# Autodesk Inventor assembly: CamLeft
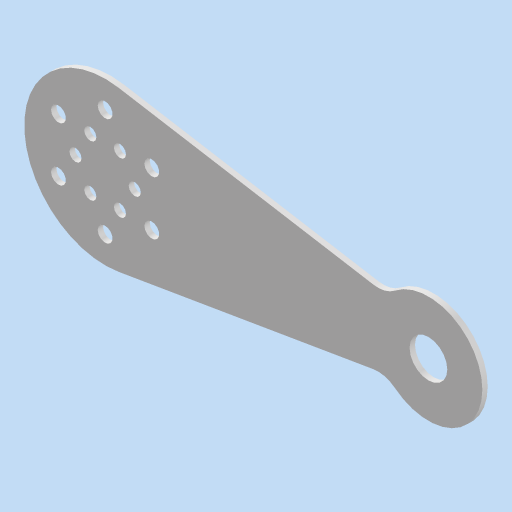
[picture p0: Inventor's stored thumbnail of the model, 512x512]
Saved by Autodesk Inventor 2023 (Build 270158000, 158)
## iProperties
Created: 2026-05-26
Part Number: CamLeft
Document SubType Name: Assembly
Designer: Nathann
Author: Nathann
Revision Number: ANY
## iProperties of the stored document MemberDocs/xCvynumyaGsfmvgzwCpa1trsjKb
Created: 2026-05-26
Part Number: CamLeft
Document SubType Name: Assembly
Designer: Nathann
Author: Nathann
Revision Number: ANY
## Documents named in this file (56)
- C:\Users\Nathann\OneDrive\ClawdDrive\Objet3D\RunningRobot\PartURDF\CamLeft.iam
- C:\Users\Nathann\OneDrive\ClawdDrive\Objet3D\RunningRobot\testfour_bar_bend_Défaut.ipt
- C:\Users\Nathann\OneDrive\ClawdDrive\Objet3D\RunningRobot\testChassis Connector.ipt
- C:\Users\Nathann\OneDrive\ClawdDrive\Objet3D\RunningRobot\testHip Hinge Base.ipt
- C:\Users\Nathann\OneDrive\ClawdDrive\Objet3D\RunningRobot\testHip Hinge Base 2.ipt
- C:\Users\Nathann\OneDrive\ClawdDrive\Objet3D\RunningRobot\testHip Motor Connector.ipt
- C:\Users\Nathann\OneDrive\ClawdDrive\Objet3D\RunningRobot\testAdduction Base.ipt
- C:\Users\Nathann\OneDrive\ClawdDrive\Objet3D\RunningRobot\testAK-60 Phantom_Défaut_1.iam
- C:\Users\Nathann\OneDrive\ClawdDrive\Objet3D\RunningRobot\testAKE90-8-KV35.ipt
- C:\Users\Nathann\OneDrive\ClawdDrive\Objet3D\RunningRobot\testDriver Placeholder.ipt
- C:\Users\Nathann\OneDrive\ClawdDrive\Objet3D\RunningRobot\testfour_bar_hip_adapter_Défaut.ipt
- C:\Users\Nathann\OneDrive\ClawdDrive\Objet3D\RunningRobot\testCFRP Tube Attachment Male Left.ipt
- C:\Users\Nathann\OneDrive\ClawdDrive\Objet3D\RunningRobot\testCFRP Tube Attachment Female_Défaut.ipt
- C:\Users\Nathann\OneDrive\ClawdDrive\Objet3D\RunningRobot\testigus adapter_Défaut.ipt
- C:\Users\Nathann\OneDrive\ClawdDrive\Objet3D\RunningRobot\testJFM-0810-05.ipt
- C:\Users\Nathann\OneDrive\ClawdDrive\Objet3D\RunningRobot\testJTM-0818-015.ipt
- C:\Users\Nathann\OneDrive\ClawdDrive\Objet3D\RunningRobot\testCFRP Tube_Défaut.ipt
- C:\Users\Nathann\OneDrive\ClawdDrive\Objet3D\RunningRobot\testCFRP Tube Attachment Male_Défaut.ipt
- C:\Users\Nathann\OneDrive\ClawdDrive\Objet3D\RunningRobot\testfour_bar_knee_adapter_Défaut.ipt
- C:\Users\Nathann\OneDrive\ClawdDrive\Objet3D\RunningRobot\testCFRP Tube Plug_Défaut.ipt
- C:\Users\Nathann\OneDrive\ClawdDrive\Objet3D\RunningRobot\testUpper Leg Plate_Défaut.ipt
- C:\Users\Nathann\OneDrive\ClawdDrive\Objet3D\RunningRobot\testUpper Leg Spacer_Défaut.ipt
- C:\Users\Nathann\OneDrive\ClawdDrive\Objet3D\RunningRobot\testMotor Adapter Plate_Défaut.ipt
- C:\Users\Nathann\OneDrive\ClawdDrive\Objet3D\RunningRobot\testKnee Joint Outer_Défaut.ipt
- C:\Users\Nathann\OneDrive\ClawdDrive\Objet3D\RunningRobot\testknee bearing holder_Défaut.ipt
- C:\Users\Nathann\OneDrive\ClawdDrive\Objet3D\RunningRobot\testShin_Spacer_Défaut.ipt
- C:\Users\Nathann\OneDrive\ClawdDrive\Objet3D\RunningRobot\testShin_Plate_Défaut.ipt
- C:\Users\Nathann\OneDrive\ClawdDrive\Objet3D\RunningRobot\testAchilles Base_Défaut.ipt
- C:\Users\Nathann\OneDrive\ClawdDrive\Objet3D\RunningRobot\testAchilles Joint_Défaut.ipt
- C:\Users\Nathann\OneDrive\ClawdDrive\Objet3D\RunningRobot\testWasher M8 ISO 7089 ALU_Défaut.ipt
- C:\Users\Nathann\OneDrive\ClawdDrive\Objet3D\RunningRobot\testNETW6.ipt
- C:\Users\Nathann\OneDrive\ClawdDrive\Objet3D\RunningRobot\testNut M8 ISO 4032_Défaut.ipt
- C:\Users\Nathann\OneDrive\ClawdDrive\Objet3D\RunningRobot\testEST-221-Durovis_EST-221-Durovis.ipt
- C:\Users\Nathann\OneDrive\ClawdDrive\Objet3D\RunningRobot\testSpring Screw Bottom_Défaut.ipt
- C:\Users\Nathann\OneDrive\ClawdDrive\Objet3D\RunningRobot\test22_1-Durovis_22_1-Durovis.ipt
- C:\Users\Nathann\OneDrive\ClawdDrive\Objet3D\RunningRobot\testCFRP Achilles_Défaut.ipt
- C:\Users\Nathann\OneDrive\ClawdDrive\Objet3D\RunningRobot\testSpring Clamp Bottom_Défaut.ipt
- C:\Users\Nathann\OneDrive\ClawdDrive\Objet3D\RunningRobot\testHeel Ext.ipt
- C:\Users\Nathann\OneDrive\ClawdDrive\Objet3D\RunningRobot\testHeel Center.ipt
- C:\Users\Nathann\OneDrive\ClawdDrive\Objet3D\RunningRobot\testFoot Spacer_Défaut.ipt
- C:\Users\Nathann\OneDrive\ClawdDrive\Objet3D\RunningRobot\testFoot Plate_Défaut.ipt
- C:\Users\Nathann\OneDrive\ClawdDrive\Objet3D\RunningRobot\testToe Connector.ipt
- C:\Users\Nathann\OneDrive\ClawdDrive\Objet3D\RunningRobot\testGGB-8_Misumi.ipt
- C:\Users\Nathann\OneDrive\ClawdDrive\Objet3D\RunningRobot\testFoot Bearing Holder_Défaut.ipt
- C:\Users\Nathann\OneDrive\ClawdDrive\Objet3D\RunningRobot\testAnkle Bearing Support 1_Défaut.ipt
- C:\Users\Nathann\OneDrive\ClawdDrive\Objet3D\RunningRobot\testAnkle Bearing Support 2_Défaut.ipt
- C:\Users\Nathann\OneDrive\ClawdDrive\Objet3D\RunningRobot\testM4x16.ipt
- C:\Users\Nathann\OneDrive\ClawdDrive\Objet3D\RunningRobot\testM3x12_Défaut.ipt
- C:\Users\Nathann\OneDrive\ClawdDrive\Objet3D\RunningRobot\testM5x20_Défaut.ipt
- C:\Users\Nathann\OneDrive\ClawdDrive\Objet3D\RunningRobot\testWasher M5 ISO 7092_Défaut.ipt
- C:\Users\Nathann\OneDrive\ClawdDrive\Objet3D\RunningRobot\testM5x50_Défaut.ipt
- C:\Users\Nathann\OneDrive\ClawdDrive\Objet3D\RunningRobot\testWasher M4 ISO 7092_Défaut.ipt
- C:\Users\Nathann\OneDrive\ClawdDrive\Objet3D\RunningRobot\testWasher M3 ISO 7092_Défaut.ipt
- C:\Users\Nathann\OneDrive\ClawdDrive\Objet3D\RunningRobot\testNut M4 DIN 985_Défaut.ipt
- C:\Users\Nathann\OneDrive\ClawdDrive\Objet3D\RunningRobot\testHülsenmutter M3x20.ipt
- C:\Users\Nathann\OneDrive\ClawdDrive\Objet3D\RunningRobot\testM3x22_Défaut.ipt
## Components (1 placed, 1 different names)
1. four_bar_bend_Défaut_22 — Mate:1, Mate:2, Mate:3
## Relationships (3: Mate 3)
- Mate:1: four_bar_bend_Défaut_22
- Mate:2: four_bar_bend_Défaut_22
- Mate:3: four_bar_bend_Défaut_22
